# Autodesk Inventor assembly: reservoir pump combo assembly
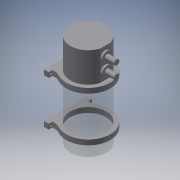
[picture p0: Inventor's stored thumbnail of the model, 180x180]
Saved by Autodesk Inventor 2018 (Build 220112000, 112)
## iProperties
Created: 2018-06-16
Part Number: reservoir pump combo assembly
Document SubType Name: Assembly
Designer: John Viljoen
Author: John Viljoen
## Documents named in this file (4)
- C:\Users\John Viljoen\Documents\Inventor\computer project\reservoir pump combo assembly.iam
- C:\Users\John Viljoen\Documents\Inventor\computer project\reservoir pump combo mount.ipt
- C:\Users\John Viljoen\Documents\Inventor\computer project\reservoir pump combo pump.ipt
- C:\Users\John Viljoen\Documents\Inventor\computer project\reservoir pump combo reservoir.ipt
## Components (4 placed, 3 different names)
1. reservoir pump combo mount:1 — Mate:4, Angle:2, Mate:6
2. reservoir pump combo mount:2 — Mate:3, Angle:1, Mate:5, Mate:6
3. reservoir pump combo pump:1 — Mate:1, Mate:2, Angle:1, Angle:2, Mate:5
4. reservoir pump combo reservoir:1 — Mate:1, Mate:2, Mate:3, Mate:4
## Relationships (8: Mate 6, Angle 2)
- Mate:1: reservoir pump combo pump:1 ↔ reservoir pump combo reservoir:1
- Mate:2: reservoir pump combo pump:1 ↔ reservoir pump combo reservoir:1
- Mate:3: reservoir pump combo mount:2 ↔ reservoir pump combo reservoir:1
- Mate:4: reservoir pump combo mount:1 ↔ reservoir pump combo reservoir:1
- Angle:1 (90 deg): reservoir pump combo mount:2 ↔ reservoir pump combo pump:1
- Angle:2 (90 deg): reservoir pump combo mount:1 ↔ reservoir pump combo pump:1
- Mate:5: reservoir pump combo mount:2 ↔ reservoir pump combo pump:1
- Mate:6 (66.6 mm): reservoir pump combo mount:1 ↔ reservoir pump combo mount:2
